# Autodesk Inventor assembly: Ensamble Final
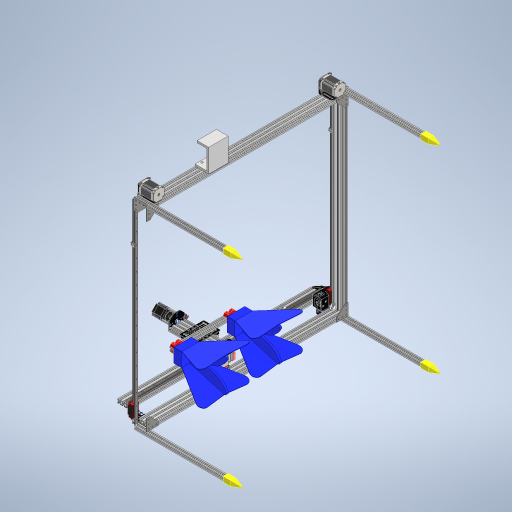
[picture p0: Inventor's stored thumbnail of the model, 512x512]
Saved by Autodesk Inventor 2024 (Build 280153000, 153)
## iProperties
Created: 2023-12-09
Part Number: Ensamble Final
Document SubType Name: Assembly
Designer: juanp
Author: juanp
## Documents named in this file (29)
- C:\Users\juanp\OneDrive - Universidad de los andes\Uniandes\GPR Portable\Ensamble de Construcción.iam
- C:\Users\juanp\OneDrive - Universidad de los andes\Uniandes\GPR Portable\Actuador\Ensamble Herramienta.iam
- C:\Users\juanp\OneDrive - Universidad de los andes\Uniandes\GPR Portable\Actuador\Actuador Lineal NEMA23\Actuador sin carro.iam
- C:\Users\juanp\OneDrive - Universidad de los andes\Uniandes\GPR Portable\Actuador\Actuador Lineal NEMA23\Carro.iam
- C:\Users\juanp\OneDrive - Universidad de los andes\Uniandes\GPR Portable\Actuador\Espaciador Actuador - Antenas.ipt
- C:\Users\juanp\OneDrive - Universidad de los andes\Uniandes\GPR Portable\Estructural\VSLOT 2060 Extrusion x 1m.ipt
- C:\Users\juanp\OneDrive - Universidad de los andes\Uniandes\GPR Portable\Estructural\Extrusion bracket.ipt
- C:\Users\juanp\OneDrive - Universidad de los andes\Uniandes\GPR Portable\Movimiento\HGH15\HGH15CA.ipt
- C:\Users\juanp\OneDrive - Universidad de los andes\Uniandes\GPR Portable\Movimiento\HGH15\HGR15R.ipt
- C:\Users\juanp\OneDrive - Universidad de los andes\Uniandes\GPR Portable\Estructural\90 Degree Cast Corner for 2020 Extrusion (Ooznest).ipt
- C:\Users\juanp\OneDrive - Universidad de los andes\Uniandes\GPR Portable\Movimiento\Motores\Stepper motor NEMA 23HS7430.ipt
- C:\Users\juanp\OneDrive - Universidad de los andes\Uniandes\GPR Portable\Estructural\Nema 23 Motor Mounting Bracket.ipt
- C:\Users\juanp\OneDrive - Universidad de los andes\Uniandes\GPR Portable\Movimiento\GT2 ID6.35 10mm.ipt
- C:\Users\juanp\OneDrive - Universidad de los andes\Uniandes\GPR Portable\Movimiento\Soporte Eje X R.ipt
- C:\Users\juanp\OneDrive - Universidad de los andes\Uniandes\GPR Portable\Actuador\Soporte Actuador Lineal.ipt
- C:\Users\juanp\OneDrive - Universidad de los andes\Uniandes\GPR Portable\Movimiento\Soporte Poleas Estaticas L.ipt
- C:\Users\juanp\OneDrive - Universidad de los andes\Uniandes\GPR Portable\Movimiento\Soporte Poleas Estaticas R.ipt
- C:\Users\juanp\OneDrive - Universidad de los andes\Uniandes\GPR Portable\Movimiento\Arandela Soporte Poleas.ipt
- C:\Users\juanp\OneDrive - Universidad de los andes\Uniandes\GPR Portable\Movimiento\Idler Pulley 10mm 5mm Bore.ipt
- C:\Users\juanp\OneDrive - Universidad de los andes\Uniandes\GPR Portable\Movimiento\Soporte Eje X L.ipt
- C:\Users\juanp\OneDrive - Universidad de los andes\Uniandes\GPR Portable\Actuador\Final de Correa.ipt
- C:\Users\juanp\OneDrive - Universidad de los andes\Uniandes\GPR Portable\Estructural\Tope Final.ipt
- C:\Users\juanp\OneDrive - Universidad de los andes\Uniandes\GPR Portable\Electrónica\Limit_switch.ipt
- C:\Users\juanp\OneDrive - Universidad de los andes\Uniandes\GPR Portable\Estructural\VSLOT 2020 Extrusion x 50cm.ipt
- C:\Users\juanp\OneDrive - Universidad de los andes\Uniandes\GPR Portable\Estructural\Pies.ipt
- C:\Users\juanp\OneDrive - Universidad de los andes\Uniandes\GPR Portable\Electrónica\Soporte Y.ipt
- C:\Users\juanp\OneDrive - Universidad de los andes\Uniandes\GPR Portable\Electrónica\Soporte X.ipt
- C:\Users\juanp\OneDrive - Universidad de los andes\Uniandes\GPR Portable\Movimiento\Suporte Switch Límite Z 2.ipt
- C:\Users\juanp\OneDrive - Universidad de los andes\Uniandes\GPR Portable\Estructural\Soporte VNA.ipt
## Components (71 placed, 28 different names)
1. Ensamble Herramienta:1 [sub-assembly] — Mate:5, Mate:6, Mate:7
2. Actuador sin carro:1 [sub-assembly] — Mate:1, Angle:1, Flush:37, Mate:56, Mate:125, Mate:131, Flush:128, Mate:140, Flush:134, Mate:141, Angle:13, Mate:143, Mate:144
3. Carro:1 [sub-assembly] — Mate:1, Angle:1, Mate:2, Mate:5, Mate:8, Mate:9
4. Espaciador Actuador - Antenas:1 — Mate:2, Mate:6, Mate:7, Mate:8, Mate:9
5. VSLOT 2060 Extrusion x 1m:1 — Mate:35, Flush:30, Angle:7, Angle:8, Flush:31, Mate:38, Mate:48, Mate:84, Mate:137, Flush:131
6. VSLOT 2060 Extrusion x 1m:2 — Flush:3, Mate:10, Flush:4, Flush:13, Flush:15, Mate:16, Mate:22, Flush:26, Mate:31, Mate:32, Angle:5, Flush:32, Flush:33, Flush:34, Flush:135, Mate:148
7. VSLOT 2060 Extrusion x 1m:3 — Flush:2, Flush:3, Mate:10, Mate:11, Flush:4, Flush:5, Flush:14, Flush:17, Flush:21, Flush:22, Mate:20, Mate:21, Flush:110, Mate:98, Mate:99
8. VSLOT 2060 Extrusion x 1m:4 — Flush:1, Flush:2, Mate:12, Flush:6, Mate:13, Flush:11, Flush:12, Mate:14, Flush:19, Flush:20, Mate:15, Mate:17, Mate:38, Flush:107, Flush:108, Mate:100, Mate:101
9. VSLOT 2060 Extrusion x 1m:5 — Flush:1, Mate:11, Flush:5, Mate:12, Flush:6, Flush:10, Flush:16, Mate:18, Mate:19, Mate:57, Mate:58, Mate:59, Mate:60
10. Extrusion bracket:1 — Flush:7, Mate:13, Flush:10, Flush:11
11. Extrusion bracket:2 — Flush:7, Flush:8, Flush:12, Flush:13
12. Extrusion bracket:3 — Flush:8, Flush:9, Flush:14, Flush:15
13. Extrusion bracket:4 — Flush:9, Flush:16, Flush:17
14. HGH15CA:1 — Flush:27, Flush:28, Mate:52, Mate:54, Mate:85, Mate:86, Mate:87, Mate:133
15. HGR15R:1 — Flush:18, Flush:21, Flush:22, Mate:52, Mate:54, Mate:126, Angle:9, Angle:10, Mate:128, Mate:130
16. HGH15CA:2 — Mate:50, Mate:51, Mate:55, Flush:35, Flush:36, Flush:132
17. HGR15R:2 — Flush:18, Mate:14, Flush:19, Flush:20, Mate:53, Angle:11, Angle:12, Mate:127, Mate:129
18. HGH15CA:3 — Flush:27, Flush:28, Angle:7, Angle:8, Mate:40, Mate:41, Mate:53, Mate:83
19. HGR15R:3 — Mate:35, Flush:30, Flush:31, Mate:50, Mate:51
20. 90 Degree Cast Corner for 2020 Extrusion (Ooznest):1 — Mate:15, Mate:16, Flush:25
21. 90 Degree Cast Corner for 2020 Extrusion (Ooznest):2 — Mate:19, Mate:20, Flush:23, Flush:24
22. 90 Degree Cast Corner for 2020 Extrusion (Ooznest):3 — Mate:21, Mate:22, Flush:23, Flush:26
23. 90 Degree Cast Corner for 2020 Extrusion (Ooznest):4 — Mate:17, Mate:18, Flush:24, Flush:25
24. Stepper motor NEMA 23HS7430:1 — Mate:25, Mate:28, Angle:3, Mate:29
25. Stepper motor NEMA 23HS7430:2 — Mate:26, Mate:27, Angle:4, Mate:30
26. Nema 23 Motor Mounting Bracket:1 — Mate:26, Mate:27, Angle:4, Flush:29, Mate:31, Flush:34, Mate:81
27. Nema 23 Motor Mounting Bracket:2 — Mate:25, Mate:28, Angle:3, Flush:29, Mate:32, Angle:5, Flush:32, Flush:33, Mate:82
28. GT2 ID6.35 10mm:1 — Mate:29, Mate:34
29. GT2 ID6.35 10mm:2 — Mate:30, Mate:34, Flush:39
30. Soporte Eje X R:1 — Mate:40, Mate:41, Mate:48, Mate:83, Mate:84, Mate:88, Flush:40
31. Soporte Actuador Lineal:1 — Mate:55, Flush:35, Flush:36, Flush:37, Mate:56, Mate:91, Mate:92, Mate:125, Mate:132, Mate:142
32. Soporte Poleas Estaticas L:1 — Mate:57, Mate:58, Mate:77, Mate:78, Mate:81
33. Soporte Poleas Estaticas R:1 — Mate:59, Mate:60, Mate:79, Mate:80, Mate:82
34. Idler Pulley 10mm 5mm Bore:1 — Mate:61, Mate:62, Mate:64, Mate:65, Mate:66
35. Arandela Soporte Poleas:2 — Mate:65, Mate:66, Mate:78
36. Arandela Soporte Poleas:3 — Mate:61, Mate:62, Mate:63
37. Arandela Soporte Poleas:5 — Mate:67, Mate:68
38. Idler Pulley 10mm 5mm Bore:3 — Mate:63, Mate:64, Mate:67, Mate:68, Mate:77, Flush:39
39. Idler Pulley 10mm 5mm Bore:4 — Mate:79
40. Arandela Soporte Poleas:6
41. Arandela Soporte Poleas:7
42. Arandela Soporte Poleas:8 — Mate:80
43. Idler Pulley 10mm 5mm Bore:5
44. Soporte Eje X L:1 — Mate:85, Mate:86, Mate:87, Mate:139
45. Final de Correa:1 — Mate:88, Flush:40, Mate:89, Mate:90, Mate:91
46. Final de Correa:2 — Mate:89, Mate:90, Mate:92
47. VSLOT 2020 Extrusion x 50cm:2 — Flush:104, Flush:105, Flush:109, Mate:101, Mate:114, Flush:113, Flush:114, Mate:123, Mate:124
48. VSLOT 2020 Extrusion x 50cm:3 — Flush:106, Flush:110, Flush:111, Mate:98, Mate:115, Flush:118, Flush:119, Mate:116, Mate:117, Mate:118
49. VSLOT 2020 Extrusion x 50cm:4 — Flush:105, Flush:106, Flush:111, Mate:99, Flush:120, Flush:121, Mate:119, Mate:120
50. VSLOT 2020 Extrusion x 50cm:5 — Flush:104, Flush:107, Flush:108, Flush:109, Mate:100, Flush:115, Flush:116, Mate:121, Mate:122
51. Extrusion bracket:5 — Flush:112, Flush:115, Flush:116
52. Extrusion bracket:6 — Flush:112, Mate:114, Flush:113, Flush:114
53. Extrusion bracket:7 — Flush:117, Flush:118, Flush:119
54. Extrusion bracket:8 — Flush:117, Mate:115, Flush:120, Flush:121
55. Pies:1 — Flush:124, Mate:116, Mate:117, Mate:118
56. Pies:2 — Flush:123, Flush:124, Mate:119, Mate:120
57. Pies:3 — Flush:122, Mate:121, Mate:122
58. Pies:4 — Flush:122, Flush:123, Mate:123, Mate:124
59. Tope Final:2 — Flush:126, Angle:9, Mate:128, Mate:133
60. Tope Final:3 — Flush:126, Flush:127, Mate:126, Angle:11, Mate:127
61. Tope Final:4 — Flush:125, Angle:10, Mate:130
62. Tope Final:5 — Flush:125, Flush:127, Angle:12, Mate:129
63. Soporte Y:1 — Mate:131, Mate:132, Flush:128, Mate:134, Mate:135, Mate:136
64. Limit_switch:1 — Mate:145, Mate:146, Mate:147
65. Limit_switch:2 — Mate:134, Mate:135, Mate:136
66. Limit_switch:3 — Mate:140, Flush:132, Flush:133
67. 90 Degree Cast Corner for 2020 Extrusion (Ooznest):5 — Flush:129, Flush:130, Flush:131, Mate:138, Mate:139
68. 90 Degree Cast Corner for 2020 Extrusion (Ooznest):6 — Flush:129, Mate:137, Flush:130, Mate:138, Flush:133
69. Soporte X:1 — Flush:134, Mate:141, Mate:142
70. Suporte Switch Límite Z 2:1 — Angle:13, Mate:143, Mate:144, Mate:145, Mate:146, Mate:147
71. Soporte VNA:1 — Flush:135, Mate:148
## Relationships (198: Mate 116, Flush 71, Angle 11)
- Mate:1: Actuador sin carro:1 ↔ Carro:1
- Angle:1 (0 deg): Actuador sin carro:1 ↔ Carro:1
- Mate:2: Carro:1 ↔ Espaciador Actuador - Antenas:1
- Mate:5: Ensamble Herramienta:1 ↔ Carro:1
- Mate:6: Ensamble Herramienta:1 ↔ Espaciador Actuador - Antenas:1
- Mate:7: Ensamble Herramienta:1 ↔ Espaciador Actuador - Antenas:1
- Mate:8: Carro:1 ↔ Espaciador Actuador - Antenas:1
- Mate:9: Carro:1 ↔ Espaciador Actuador - Antenas:1
- Flush:1: VSLOT 2060 Extrusion x 1m:4 ↔ VSLOT 2060 Extrusion x 1m:5
- Flush:2: VSLOT 2060 Extrusion x 1m:3 ↔ VSLOT 2060 Extrusion x 1m:4
- Flush:3: VSLOT 2060 Extrusion x 1m:2 ↔ VSLOT 2060 Extrusion x 1m:3
- Mate:10: VSLOT 2060 Extrusion x 1m:2 ↔ VSLOT 2060 Extrusion x 1m:3
- Mate:11: VSLOT 2060 Extrusion x 1m:3 ↔ VSLOT 2060 Extrusion x 1m:5
- Flush:4: VSLOT 2060 Extrusion x 1m:2 ↔ VSLOT 2060 Extrusion x 1m:3
- Flush:5: VSLOT 2060 Extrusion x 1m:3 ↔ VSLOT 2060 Extrusion x 1m:5
- Mate:12: VSLOT 2060 Extrusion x 1m:4 ↔ VSLOT 2060 Extrusion x 1m:5
- Flush:6: VSLOT 2060 Extrusion x 1m:4 ↔ VSLOT 2060 Extrusion x 1m:5
- Flush:7: Extrusion bracket:1 ↔ Extrusion bracket:2
- Flush:8: Extrusion bracket:2 ↔ Extrusion bracket:3
- Flush:9: Extrusion bracket:3 ↔ Extrusion bracket:4
- Mate:13: VSLOT 2060 Extrusion x 1m:4 ↔ Extrusion bracket:1
- Flush:10: VSLOT 2060 Extrusion x 1m:5 ↔ Extrusion bracket:1
- Flush:11: VSLOT 2060 Extrusion x 1m:4 ↔ Extrusion bracket:1
- Flush:12: VSLOT 2060 Extrusion x 1m:4 ↔ Extrusion bracket:2
- Flush:13: VSLOT 2060 Extrusion x 1m:2 ↔ Extrusion bracket:2
- Flush:14: VSLOT 2060 Extrusion x 1m:3 ↔ Extrusion bracket:3
- Flush:15: VSLOT 2060 Extrusion x 1m:2 ↔ Extrusion bracket:3
- Flush:16: VSLOT 2060 Extrusion x 1m:5 ↔ Extrusion bracket:4
- Flush:17: VSLOT 2060 Extrusion x 1m:3 ↔ Extrusion bracket:4
- Flush:18: HGR15R:1 ↔ HGR15R:2
- Mate:14: VSLOT 2060 Extrusion x 1m:4 ↔ HGR15R:2
- Flush:19: VSLOT 2060 Extrusion x 1m:4 ↔ HGR15R:2
- Flush:20 (2.5 mm): VSLOT 2060 Extrusion x 1m:4 ↔ HGR15R:2
- Flush:21: VSLOT 2060 Extrusion x 1m:3 ↔ HGR15R:1
- Flush:22 (2.5 mm): VSLOT 2060 Extrusion x 1m:3 ↔ HGR15R:1
- Mate:15: VSLOT 2060 Extrusion x 1m:4 ↔ 90 Degree Cast Corner for 2020 Extrusion (Ooznest):1
- Mate:16: VSLOT 2060 Extrusion x 1m:2 ↔ 90 Degree Cast Corner for 2020 Extrusion (Ooznest):1
- Mate:17: VSLOT 2060 Extrusion x 1m:4 ↔ 90 Degree Cast Corner for 2020 Extrusion (Ooznest):4
- Mate:18: VSLOT 2060 Extrusion x 1m:5 ↔ 90 Degree Cast Corner for 2020 Extrusion (Ooznest):4
- Mate:19: VSLOT 2060 Extrusion x 1m:5 ↔ 90 Degree Cast Corner for 2020 Extrusion (Ooznest):2
- Mate:20: VSLOT 2060 Extrusion x 1m:3 ↔ 90 Degree Cast Corner for 2020 Extrusion (Ooznest):2
- Mate:21: VSLOT 2060 Extrusion x 1m:3 ↔ 90 Degree Cast Corner for 2020 Extrusion (Ooznest):3
- Mate:22: VSLOT 2060 Extrusion x 1m:2 ↔ 90 Degree Cast Corner for 2020 Extrusion (Ooznest):3
- Flush:23: 90 Degree Cast Corner for 2020 Extrusion (Ooznest):2 ↔ 90 Degree Cast Corner for 2020 Extrusion (Ooznest):3
- Flush:24: 90 Degree Cast Corner for 2020 Extrusion (Ooznest):2 ↔ 90 Degree Cast Corner for 2020 Extrusion (Ooznest):4
- Flush:25: 90 Degree Cast Corner for 2020 Extrusion (Ooznest):1 ↔ 90 Degree Cast Corner for 2020 Extrusion (Ooznest):4
- Flush:26 (10 mm): VSLOT 2060 Extrusion x 1m:2 ↔ 90 Degree Cast Corner for 2020 Extrusion (Ooznest):3
- Flush:27: HGH15CA:1 ↔ HGH15CA:3
- Flush:28: HGH15CA:1 ↔ HGH15CA:3
- Mate:25: Stepper motor NEMA 23HS7430:1 ↔ Nema 23 Motor Mounting Bracket:2
- Mate:26: Stepper motor NEMA 23HS7430:2 ↔ Nema 23 Motor Mounting Bracket:1
- Mate:27: Stepper motor NEMA 23HS7430:2 ↔ Nema 23 Motor Mounting Bracket:1
- Mate:28: Stepper motor NEMA 23HS7430:1 ↔ Nema 23 Motor Mounting Bracket:2
- Angle:3 (0 deg): Stepper motor NEMA 23HS7430:1 ↔ Nema 23 Motor Mounting Bracket:2
- Angle:4 (0 deg): Stepper motor NEMA 23HS7430:2 ↔ Nema 23 Motor Mounting Bracket:1
- Mate:29: Stepper motor NEMA 23HS7430:1 ↔ GT2 ID6.35 10mm:1
- Mate:30: Stepper motor NEMA 23HS7430:2 ↔ GT2 ID6.35 10mm:2
- Flush:29: Nema 23 Motor Mounting Bracket:1 ↔ Nema 23 Motor Mounting Bracket:2
- Mate:31: VSLOT 2060 Extrusion x 1m:2 ↔ Nema 23 Motor Mounting Bracket:1
- Mate:32: VSLOT 2060 Extrusion x 1m:2 ↔ Nema 23 Motor Mounting Bracket:2
- Mate:34 (-3 mm): GT2 ID6.35 10mm:1 ↔ GT2 ID6.35 10mm:2
- Angle:5 (0 deg): VSLOT 2060 Extrusion x 1m:2 ↔ Nema 23 Motor Mounting Bracket:2
- Mate:35: VSLOT 2060 Extrusion x 1m:1 ↔ HGR15R:3
- Flush:30: VSLOT 2060 Extrusion x 1m:1 ↔ HGR15R:3
- Angle:7 (0 deg): VSLOT 2060 Extrusion x 1m:1 ↔ HGH15CA:3
- Angle:8 (180 deg): VSLOT 2060 Extrusion x 1m:1 ↔ HGH15CA:3
- Flush:31 (2.5 mm): VSLOT 2060 Extrusion x 1m:1 ↔ HGR15R:3
- Mate:38: VSLOT 2060 Extrusion x 1m:1 ↔ VSLOT 2060 Extrusion x 1m:4
- Flush:32 (-5 mm): VSLOT 2060 Extrusion x 1m:2 ↔ Nema 23 Motor Mounting Bracket:2
- Flush:33: VSLOT 2060 Extrusion x 1m:2 ↔ Nema 23 Motor Mounting Bracket:2
- Flush:34: VSLOT 2060 Extrusion x 1m:2 ↔ Nema 23 Motor Mounting Bracket:1
- Mate:40: HGH15CA:3 ↔ Soporte Eje X R:1
- Mate:41: HGH15CA:3 ↔ Soporte Eje X R:1
- Mate:48: VSLOT 2060 Extrusion x 1m:1 ↔ Soporte Eje X R:1
- Mate:50: HGH15CA:2 ↔ HGR15R:3
- Mate:51: HGH15CA:2 ↔ HGR15R:3
- Mate:52: HGH15CA:1 ↔ HGR15R:1
- Mate:53: HGR15R:2 ↔ HGH15CA:3
- Mate:54: HGH15CA:1 ↔ HGR15R:1
- Mate:55: HGH15CA:2 ↔ Soporte Actuador Lineal:1
- Flush:35: HGH15CA:2 ↔ Soporte Actuador Lineal:1
- Flush:36: HGH15CA:2 ↔ Soporte Actuador Lineal:1
- Flush:37: Actuador sin carro:1 ↔ Soporte Actuador Lineal:1
- Mate:56: Actuador sin carro:1 ↔ Soporte Actuador Lineal:1
- Mate:57: VSLOT 2060 Extrusion x 1m:5 ↔ Soporte Poleas Estaticas L:1
- Mate:58: VSLOT 2060 Extrusion x 1m:5 ↔ Soporte Poleas Estaticas L:1
- Mate:59: VSLOT 2060 Extrusion x 1m:5 ↔ Soporte Poleas Estaticas R:1
- Mate:60: VSLOT 2060 Extrusion x 1m:5 ↔ Soporte Poleas Estaticas R:1
- Mate:61: Idler Pulley 10mm 5mm Bore:1 ↔ Arandela Soporte Poleas:3
- Mate:62: Idler Pulley 10mm 5mm Bore:1 ↔ Arandela Soporte Poleas:3
- Mate:63: Arandela Soporte Poleas:3 ↔ Idler Pulley 10mm 5mm Bore:3
- Mate:64: Idler Pulley 10mm 5mm Bore:1 ↔ Idler Pulley 10mm 5mm Bore:3
- Mate:65: Idler Pulley 10mm 5mm Bore:1 ↔ Arandela Soporte Poleas:2
- Mate:66: Idler Pulley 10mm 5mm Bore:1 ↔ Arandela Soporte Poleas:2
- Mate:67: Arandela Soporte Poleas:5 ↔ Idler Pulley 10mm 5mm Bore:3
- Mate:68: Arandela Soporte Poleas:5 ↔ Idler Pulley 10mm 5mm Bore:3
- [Mate]: Idler Pulley 10mm 5mm Bore:4 ↔ Arandela Soporte Poleas:7
- [Mate]: Idler Pulley 10mm 5mm Bore:4 ↔ Arandela Soporte Poleas:7
- [Mate]: Arandela Soporte Poleas:7 ↔ Idler Pulley 10mm 5mm Bore:5
- [Mate]: Idler Pulley 10mm 5mm Bore:4 ↔ Idler Pulley 10mm 5mm Bore:5
- [Mate]: Idler Pulley 10mm 5mm Bore:4 ↔ Arandela Soporte Poleas:6
- [Mate]: Idler Pulley 10mm 5mm Bore:4 ↔ Arandela Soporte Poleas:6
- [Mate]: Arandela Soporte Poleas:8 ↔ Idler Pulley 10mm 5mm Bore:5
- [Mate]: Arandela Soporte Poleas:8 ↔ Idler Pulley 10mm 5mm Bore:5
- Mate:77: Soporte Poleas Estaticas L:1 ↔ Idler Pulley 10mm 5mm Bore:3
- Mate:78: Soporte Poleas Estaticas L:1 ↔ Arandela Soporte Poleas:2
- Mate:79: Soporte Poleas Estaticas R:1 ↔ Idler Pulley 10mm 5mm Bore:4
- Mate:80: Soporte Poleas Estaticas R:1 ↔ Arandela Soporte Poleas:8
- Flush:39: GT2 ID6.35 10mm:2 ↔ Idler Pulley 10mm 5mm Bore:3
- Mate:81: Nema 23 Motor Mounting Bracket:1 ↔ Soporte Poleas Estaticas L:1
- Mate:82: Nema 23 Motor Mounting Bracket:2 ↔ Soporte Poleas Estaticas R:1
- Mate:83: HGH15CA:3 ↔ Soporte Eje X R:1
- Mate:84: VSLOT 2060 Extrusion x 1m:1 ↔ Soporte Eje X R:1
- Mate:85: HGH15CA:1 ↔ Soporte Eje X L:1
- Mate:86: HGH15CA:1 ↔ Soporte Eje X L:1
- Mate:87: HGH15CA:1 ↔ Soporte Eje X L:1
- Mate:88: Soporte Eje X R:1 ↔ Final de Correa:1
- Flush:40: Soporte Eje X R:1 ↔ Final de Correa:1
- Mate:89: Final de Correa:1 ↔ Final de Correa:2
- Mate:90: Final de Correa:1 ↔ Final de Correa:2
- Mate:91 (10 mm): Soporte Actuador Lineal:1 ↔ Final de Correa:1
- Mate:92 (10 mm): Soporte Actuador Lineal:1 ↔ Final de Correa:2
- Flush:104: VSLOT 2020 Extrusion x 50cm:2 ↔ VSLOT 2020 Extrusion x 50cm:5
- Flush:105: VSLOT 2020 Extrusion x 50cm:2 ↔ VSLOT 2020 Extrusion x 50cm:4
- Flush:106: VSLOT 2020 Extrusion x 50cm:3 ↔ VSLOT 2020 Extrusion x 50cm:4
- Flush:107: VSLOT 2060 Extrusion x 1m:4 ↔ VSLOT 2020 Extrusion x 50cm:5
- Flush:108: VSLOT 2060 Extrusion x 1m:4 ↔ VSLOT 2020 Extrusion x 50cm:5
- Flush:109: VSLOT 2020 Extrusion x 50cm:2 ↔ VSLOT 2020 Extrusion x 50cm:5
- Flush:110: VSLOT 2060 Extrusion x 1m:3 ↔ VSLOT 2020 Extrusion x 50cm:3
- Flush:111: VSLOT 2020 Extrusion x 50cm:3 ↔ VSLOT 2020 Extrusion x 50cm:4
- Mate:98: VSLOT 2060 Extrusion x 1m:3 ↔ VSLOT 2020 Extrusion x 50cm:3
- Mate:99: VSLOT 2060 Extrusion x 1m:3 ↔ VSLOT 2020 Extrusion x 50cm:4
- Mate:100: VSLOT 2060 Extrusion x 1m:4 ↔ VSLOT 2020 Extrusion x 50cm:5
- Mate:101: VSLOT 2060 Extrusion x 1m:4 ↔ VSLOT 2020 Extrusion x 50cm:2
- Flush:112: Extrusion bracket:5 ↔ Extrusion bracket:6
- Mate:114: VSLOT 2020 Extrusion x 50cm:2 ↔ Extrusion bracket:6
- Flush:113: VSLOT 2020 Extrusion x 50cm:2 ↔ Extrusion bracket:6
- Flush:114: VSLOT 2020 Extrusion x 50cm:2 ↔ Extrusion bracket:6
- Flush:115: VSLOT 2020 Extrusion x 50cm:5 ↔ Extrusion bracket:5
- Flush:116: VSLOT 2020 Extrusion x 50cm:5 ↔ Extrusion bracket:5
- Flush:117: Extrusion bracket:7 ↔ Extrusion bracket:8
- Mate:115: VSLOT 2020 Extrusion x 50cm:3 ↔ Extrusion bracket:8
- Flush:118: VSLOT 2020 Extrusion x 50cm:3 ↔ Extrusion bracket:7
- Flush:119: VSLOT 2020 Extrusion x 50cm:3 ↔ Extrusion bracket:7
- Flush:120: VSLOT 2020 Extrusion x 50cm:4 ↔ Extrusion bracket:8
- Flush:121: VSLOT 2020 Extrusion x 50cm:4 ↔ Extrusion bracket:8
- Flush:122: Pies:3 ↔ Pies:4
- Flush:123: Pies:2 ↔ Pies:4
- Flush:124: Pies:1 ↔ Pies:2
- Mate:116: VSLOT 2020 Extrusion x 50cm:3 ↔ Pies:1
- Mate:117: VSLOT 2020 Extrusion x 50cm:3 ↔ Pies:1
- Mate:118: VSLOT 2020 Extrusion x 50cm:3 ↔ Pies:1
- Mate:119: VSLOT 2020 Extrusion x 50cm:4 ↔ Pies:2
- Mate:120: VSLOT 2020 Extrusion x 50cm:4 ↔ Pies:2
- Mate:121: VSLOT 2020 Extrusion x 50cm:5 ↔ Pies:3
- Mate:122: VSLOT 2020 Extrusion x 50cm:5 ↔ Pies:3
- Mate:123: VSLOT 2020 Extrusion x 50cm:2 ↔ Pies:4
- Mate:124: VSLOT 2020 Extrusion x 50cm:2 ↔ Pies:4
- Mate:125 (12.5 mm): Actuador sin carro:1 ↔ Soporte Actuador Lineal:1
- Flush:125: Tope Final:4 ↔ Tope Final:5
- Flush:126: Tope Final:2 ↔ Tope Final:3
- Flush:127: Tope Final:3 ↔ Tope Final:5
- Mate:126: HGR15R:1 ↔ Tope Final:3
- Angle:9 (0 deg): HGR15R:1 ↔ Tope Final:2
- Angle:10 (0 deg): HGR15R:1 ↔ Tope Final:4
- Angle:11 (0 deg): HGR15R:2 ↔ Tope Final:3
- Angle:12 (0 deg): HGR15R:2 ↔ Tope Final:5
- Mate:127: HGR15R:2 ↔ Tope Final:3
- Mate:128: HGR15R:1 ↔ Tope Final:2
- Mate:129: HGR15R:2 ↔ Tope Final:5
- Mate:130: HGR15R:1 ↔ Tope Final:4
- Mate:131: Actuador sin carro:1 ↔ Soporte Y:1
- Mate:132: Soporte Actuador Lineal:1 ↔ Soporte Y:1
- Flush:128: Actuador sin carro:1 ↔ Soporte Y:1
- Mate:133: HGH15CA:1 ↔ Tope Final:2
- Mate:134: Soporte Y:1 ↔ Limit_switch:2
- Mate:135: Soporte Y:1 ↔ Limit_switch:2
- Mate:136: Soporte Y:1 ↔ Limit_switch:2
- Flush:129: 90 Degree Cast Corner for 2020 Extrusion (Ooznest):5 ↔ 90 Degree Cast Corner for 2020 Extrusion (Ooznest):6
- Mate:137: VSLOT 2060 Extrusion x 1m:1 ↔ 90 Degree Cast Corner for 2020 Extrusion (Ooznest):6
- Flush:130: 90 Degree Cast Corner for 2020 Extrusion (Ooznest):5 ↔ 90 Degree Cast Corner for 2020 Extrusion (Ooznest):6
- Flush:131 (20 mm): VSLOT 2060 Extrusion x 1m:1 ↔ 90 Degree Cast Corner for 2020 Extrusion (Ooznest):5
- Mate:138 (600 mm): 90 Degree Cast Corner for 2020 Extrusion (Ooznest):5 ↔ 90 Degree Cast Corner for 2020 Extrusion (Ooznest):6
- Mate:139 (200 mm): Soporte Eje X L:1 ↔ 90 Degree Cast Corner for 2020 Extrusion (Ooznest):5
- Mate:140 (30 mm): Actuador sin carro:1 ↔ Limit_switch:3
- Flush:132: HGH15CA:2 ↔ Limit_switch:3
- Flush:133 (10 mm): Limit_switch:3 ↔ 90 Degree Cast Corner for 2020 Extrusion (Ooznest):6
- Flush:134 (20 mm): Actuador sin carro:1 ↔ Soporte X:1
- Mate:141: Actuador sin carro:1 ↔ Soporte X:1
- Mate:142: Soporte Actuador Lineal:1 ↔ Soporte X:1
- Angle:13 (0 deg): Actuador sin carro:1 ↔ Suporte Switch Límite Z 2:1
- Mate:143 (-10 mm): Actuador sin carro:1 ↔ Suporte Switch Límite Z 2:1
- Mate:144: Actuador sin carro:1 ↔ Suporte Switch Límite Z 2:1
- Mate:145: Limit_switch:1 ↔ Suporte Switch Límite Z 2:1
- Mate:146: Limit_switch:1 ↔ Suporte Switch Límite Z 2:1
- Mate:147 (3 mm): Limit_switch:1 ↔ Suporte Switch Límite Z 2:1
- Flush:135: VSLOT 2060 Extrusion x 1m:2 ↔ Soporte VNA:1
- Mate:148: VSLOT 2060 Extrusion x 1m:2 ↔ Soporte VNA:1
## Named parameters: d123_d115 = 0 mm, d124_d116 = 0 mm, d125_d117 = 0 mm, d126_d118 = 0 mm, d127_d119 = 0 mm, d128_d120 = 0 mm, d129_d121 = 0 mm, d130_d122 = 0 mm
